# Autodesk Inventor assembly: Vibrationsdaempfer_Einheit
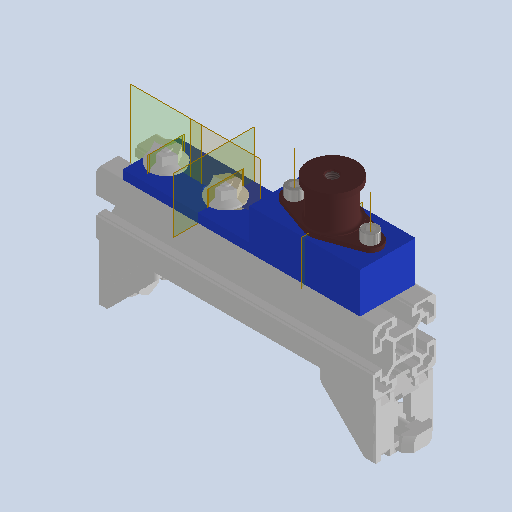
[picture p0: Inventor's stored thumbnail of the model, 512x512]
Saved by Autodesk Inventor 2025.2 (Build 292293000, 293)
## iProperties
Created: 2025-06-22
Part Number: Vibrationsdaempfer_Einheit
Document SubType Name: Assembly
Designer: Jakob
Author: Jakob
## Documents named in this file (9)
- C:\Users\tino\Documents_VM\Konstruieren_CAD\Useless Box\Eigene Bauteile\Vibrationsdaempfer\Vibrationsdaempfer_Einheit.iam
- C:\Users\tino\Documents_VM\Konstruieren_CAD\Useless Box\Eigene Bauteile\Vibrationsdaempfer\Rexroth_Profil_40x40_2175_8.ipt
- C:\Users\tino\Documents_VM\Konstruieren_CAD\Useless Box\Kaufteile\Winkel_Rexroth_40x40\Rexroth_Winkel_40x40_3D_203_MIR.iam
- C:\Users\tino\Documents_VM\Konstruieren_CAD\Useless Box\Eigene Bauteile\Vibrationsdaempfer\Adapterplatte_Vibrationsdaempfer.ipt
- C:\Users\tino\Documents_VM\Konstruieren_CAD\Useless Box\Eigene Bauteile\Vibrationsdaempfer\AIS2024\NHF19-3026-M8.ipt
- C:\Users\tino\Documents_VM\Konstruieren_CAD\Useless Box\Standart Bauteile\ISO 4762 - M6 x 12ISO.ipt
- C:\Users\Jakob\Documents\Inventor\Content Center Files\R2025\de-DE\ISO 4762(1)\DIN EN ISO 4762 - M8 x 16.ipt
- C:\Users\Jakob\Documents\Inventor\Content Center Files\R2025\de-DE\DIN 125-1  A\DIN 125 - A 8,4.ipt
- C:\Users\tino\Documents_VM\Konstruieren_CAD\Useless Box\Eigene Bauteile\Vibrationsdaempfer\Rexroth_Schraube_Mutter_modifiziert_fuer_daempfer.iam
## Components (11 placed, 8 different names)
1. Rexroth_Profil_40x40_2175_8:1 — Passend:1, Passend:2, Fluchtend:1, Passend:3, Fluchtend:3, Passend:4, Passend:6, Fluchtend:4, Passend:10
2. Rexroth_Winkel_40x40_3D_203_MIR:1 [sub-assembly] — Passend:3, Fluchtend:2, Fluchtend:3
3. Rexroth_Winkel_40x40_3D_203_MIR:2 [sub-assembly] — Passend:4, Passend:5, Passend:6
4. Adapterplatte_Vibrationsdaempfer:1 — Passend:7, Fluchtend:4, Fluchtend:6, Passend:8, Passend:9, Passend:20, Passend:21, Winkel:1, Passend:22, Passend:23, Fluchtend:7
5. NHF19-3026-M8:1 — Fluchtend:6, Passend:8, Passend:9, Passend:10, Passend:11, Passend:12, Passend:13, Passend:14, Passend:15, Passend:18
6. ISO 4762 - M6 x 12ISO:1 — Passend:12, Passend:14
7. ISO 4762 - M6 x 12ISO:2 — Passend:11, Passend:13
8. DIN EN ISO 4762 M8 x 16:1 — Passend:15, Passend:16, Passend:17
9. DIN 125-1 A A 8,4:1 — Passend:16, Passend:17, Passend:18
10. Rexroth_Schraube_Mutter_modifiziert_fuer_daempfer:1 [sub-assembly] — Passend:22, Passend:23, Fluchtend:7
11. Rexroth_Schraube_Mutter_modifiziert_fuer_daempfer:2 [sub-assembly] — Passend:20, Passend:21, Winkel:1
## Relationships (29: Mate 22, Flush 6, Angle 1)
- Passend:1 [Mate]: Rexroth_Profil_40x40_2175_8:1
- Passend:2 [Mate]: Rexroth_Profil_40x40_2175_8:1
- Fluchtend:1 [Flush]: Rexroth_Profil_40x40_2175_8:1
- Passend:3 [Mate]: Rexroth_Profil_40x40_2175_8:1 ↔ Rexroth_Winkel_40x40_3D_203_MIR:1
- Fluchtend:2 [Flush]: Rexroth_Winkel_40x40_3D_203_MIR:1
- Fluchtend:3 [Flush]: Rexroth_Profil_40x40_2175_8:1 ↔ Rexroth_Winkel_40x40_3D_203_MIR:1
- Passend:4 [Mate]: Rexroth_Profil_40x40_2175_8:1 ↔ Rexroth_Winkel_40x40_3D_203_MIR:2
- Passend:5 [Mate]: Rexroth_Winkel_40x40_3D_203_MIR:2
- Passend:6 [Mate]: Rexroth_Profil_40x40_2175_8:1 ↔ Rexroth_Winkel_40x40_3D_203_MIR:2
- Passend:7 [Mate]: Adapterplatte_Vibrationsdaempfer:1
- Fluchtend:4 [Flush]: Rexroth_Profil_40x40_2175_8:1 ↔ Adapterplatte_Vibrationsdaempfer:1
- Fluchtend:6 [Flush]: Adapterplatte_Vibrationsdaempfer:1 ↔ NHF19-3026-M8:1
- Passend:8 [Mate]: Adapterplatte_Vibrationsdaempfer:1 ↔ NHF19-3026-M8:1
- Passend:9 [Mate]: Adapterplatte_Vibrationsdaempfer:1 ↔ NHF19-3026-M8:1
- Passend:10 [Mate] (45.642 mm): Rexroth_Profil_40x40_2175_8:1 ↔ NHF19-3026-M8:1
- Passend:11 [Mate]: NHF19-3026-M8:1 ↔ ISO 4762 - M6 x 12ISO:2
- Passend:12 [Mate]: NHF19-3026-M8:1 ↔ ISO 4762 - M6 x 12ISO:1
- Passend:13 [Mate]: NHF19-3026-M8:1 ↔ ISO 4762 - M6 x 12ISO:2
- Passend:14 [Mate]: NHF19-3026-M8:1 ↔ ISO 4762 - M6 x 12ISO:1
- Passend:15 [Mate]: NHF19-3026-M8:1 ↔ DIN EN ISO 4762 M8 x 16:1
- Passend:16 [Mate]: DIN EN ISO 4762 M8 x 16:1 ↔ DIN 125-1 A A 8,4:1
- Passend:17 [Mate]: DIN EN ISO 4762 M8 x 16:1 ↔ DIN 125-1 A A 8,4:1
- Passend:18 [Mate] (5.0109 mm): NHF19-3026-M8:1 ↔ DIN 125-1 A A 8,4:1
- Passend:20 [Mate]: Adapterplatte_Vibrationsdaempfer:1 ↔ Rexroth_Schraube_Mutter_modifiziert_fuer_daempfer:2
- Passend:21 [Mate]: Adapterplatte_Vibrationsdaempfer:1 ↔ Rexroth_Schraube_Mutter_modifiziert_fuer_daempfer:2
- Winkel:1 [Angle] (0 deg): Adapterplatte_Vibrationsdaempfer:1 ↔ Rexroth_Schraube_Mutter_modifiziert_fuer_daempfer:2
- Passend:22 [Mate]: Adapterplatte_Vibrationsdaempfer:1 ↔ Rexroth_Schraube_Mutter_modifiziert_fuer_daempfer:1
- Passend:23 [Mate]: Adapterplatte_Vibrationsdaempfer:1 ↔ Rexroth_Schraube_Mutter_modifiziert_fuer_daempfer:1
- Fluchtend:7 [Flush]: Adapterplatte_Vibrationsdaempfer:1 ↔ Rexroth_Schraube_Mutter_modifiziert_fuer_daempfer:1
